# Autodesk Inventor assembly: SingleSide
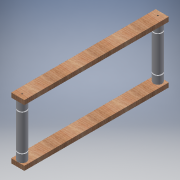
[picture p0: Inventor's stored thumbnail of the model, 180x180]
Saved by Autodesk Inventor 2016 (Build 200138000, 138)
## iProperties
Created: 2016-01-18
Part Number: SingleSide
Document SubType Name: Assembly
Designer: yash
Author: yash
## Documents named in this file (4)
- C:\Users\yash\Documents\GitHub\Robotics2016\CAD\LowGoal\PickupPrototype0\SingleSide.iam
- C:\Users\yash\Documents\GitHub\Robotics2016\CAD\LowGoal\PickupPrototype0\CarrierBracket.ipt
- C:\Users\yash\Documents\GitHub\Robotics2016\CAD\LowGoal\PickupPrototype0\Roller.ipt
- C:\Users\yash\Documents\GitHub\Robotics2016\CAD\LowGoal\PickupPrototype0\StatorShaft.ipt
## Components (6 placed, 3 different names)
1. CarrierBracket:1 — Mate:1, Mate:2, Flush:1, Flush:2
2. Roller:1 — Insert:1
3. StatorShaft:1 — Mate:1, Flush:2, Insert:1, Insert:3
4. Roller:2 — Insert:2
5. StatorShaft:2 — Mate:2, Flush:1, Insert:2, Insert:4
6. CarrierBracket:2 — Insert:3, Insert:4
## Relationships (8: Insert 4, Mate 2, Flush 2)
- Mate:1: CarrierBracket:1 ↔ StatorShaft:1
- Mate:2: CarrierBracket:1 ↔ StatorShaft:2
- Flush:1: CarrierBracket:1 ↔ StatorShaft:2
- Flush:2: CarrierBracket:1 ↔ StatorShaft:1
- Insert:1 (-25.4 mm): Roller:1 ↔ StatorShaft:1
- Insert:2 (-25.4 mm): Roller:2 ↔ StatorShaft:2
- Insert:3: StatorShaft:1 ↔ CarrierBracket:2
- Insert:4: StatorShaft:2 ↔ CarrierBracket:2
